# Autodesk Inventor assembly: Monitor with Plug Assembly
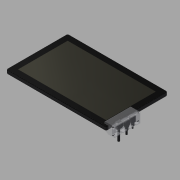
[picture p0: Inventor's stored thumbnail of the model, 180x180]
Saved by Autodesk Inventor 2019 (Build 230136000, 136)
## iProperties
Created: 2019-02-12
Part Number: Monitor with Plug Assembly
Document SubType Name: Assembly
Designer: Ben
Author: Ben
## Documents named in this file (5)
- C:\Users\Ben\Documents\Inventor\HydraVivarium\Monitor with Plug Assembly.iam
- C:\Users\Ben\Documents\Inventor\HydraVivarium\Monitor with Plugs.iam
- C:\Users\Ben\Documents\Inventor\HydraVivarium\Plug Protection Block.ipt
- C:\Users\Ben\Documents\Inventor\HydraVivarium\Plug Protection Block Insert.ipt
- C:\Users\Ben\Documents\Inventor\HydraVivarium\M1.7_6mm self-tapping screw.ipt
## Components (7 placed, 4 different names)
1. Monitor with Plugs:1 [sub-assembly] — Mate:2, Angle:2, Angle:4, Mate:3
2. Plug Protection Block:1 — Mate:1, Angle:1, Angle:2, Angle:3, Angle:4, Flush:1, Mate:3, Insert:1, Insert:2, Insert:3, Insert:4
3. Plug Protection Block Insert:1 — Mate:1, Angle:1, Mate:2, Angle:3, Flush:1
4. M1.7_6mm self-tapping screw:1 — Insert:2
5. M1.7_6mm self-tapping screw:2 — Insert:1
6. M1.7_6mm self-tapping screw:3 — Insert:3
7. M1.7_6mm self-tapping screw:4 — Insert:4
## Relationships (12: Angle 4, Insert 4, Mate 3, Flush 1)
- Mate:1: Plug Protection Block:1 ↔ Plug Protection Block Insert:1
- Angle:1 (0 deg): Plug Protection Block:1 ↔ Plug Protection Block Insert:1
- Mate:2: Monitor with Plugs:1 ↔ Plug Protection Block Insert:1
- Angle:2 (0 deg): Monitor with Plugs:1 ↔ Plug Protection Block:1
- Angle:3 (0 deg): Plug Protection Block:1 ↔ Plug Protection Block Insert:1
- Angle:4 (180 deg): Monitor with Plugs:1 ↔ Plug Protection Block:1
- Flush:1: Plug Protection Block:1 ↔ Plug Protection Block Insert:1
- Mate:3 (0.25 mm): Monitor with Plugs:1 ↔ Plug Protection Block:1
- Insert:1: Plug Protection Block:1 ↔ M1.7_6mm self-tapping screw:2
- Insert:2: Plug Protection Block:1 ↔ M1.7_6mm self-tapping screw:1
- Insert:3: Plug Protection Block:1 ↔ M1.7_6mm self-tapping screw:3
- Insert:4: Plug Protection Block:1 ↔ M1.7_6mm self-tapping screw:4
